# Autodesk Inventor assembly: Pump_V3
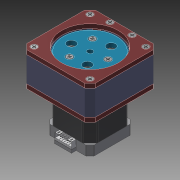
[picture p0: Inventor's stored thumbnail of the model, 180x180]
Saved by Autodesk Inventor 2022 (Build 260153000, 153)
## iProperties
Created: 2025-01-26
Part Number: Pump_V3
Document SubType Name: Assembly
Designer: Ivan
Author: Ivan
## Documents named in this file (11)
- E:\4. Прочее\1517\Предпрофессиональная олимпиада\Насос\Itteration_4\Pump_V4.iam
- E:\4. Прочее\1517\Предпрофессиональная олимпиада\Насос\Itteration_4\Nema_17.ipt
- E:\4. Прочее\1517\Предпрофессиональная олимпиада\Насос\Itteration_4\Pump_V3_Основание.ipt
- E:\4. Прочее\1517\Предпрофессиональная олимпиада\Насос\Itteration_4\ISO 7046-1 - M3 x 8_ - 4.8 - H - ISO.ipt
- E:\4. Прочее\1517\Предпрофессиональная олимпиада\Насос\Itteration_4\Pump_V3_Полумуфта.ipt
- E:\4. Прочее\1517\Предпрофессиональная олимпиада\Насос\Itteration_4\Abec 7 608 zz.ipt
- E:\4. Прочее\1517\Предпрофессиональная олимпиада\Насос\Itteration_4\Pump_V3_Втулка.ipt
- E:\4. Прочее\1517\Предпрофессиональная олимпиада\Насос\Itteration_4\Втулка Впаиваемая М3х4.2х5.ipt
- E:\4. Прочее\1517\Предпрофессиональная олимпиада\Насос\Itteration_4\ISO 7046-1 - M3 x 20_ - 4.8 - H - ISO.ipt
- E:\4. Прочее\1517\Предпрофессиональная олимпиада\Насос\Itteration_4\Pump_V4_Корпус.iam
- E:\4. Прочее\1517\Предпрофессиональная олимпиада\Насос\Itteration_4\Pump_V4_Крышка.ipt
## Components (34 placed, 10 different names)
1. Nema_17:1 — Совмещение:1, Совмещение:2, Совмещение:3, Совмещение:5
2. Pump_V3_Основание:1 — Совмещение:1, Совмещение:2, Совмещение:3, Совмещение:4, Заподлицо:1, Совмещение:6, Совмещение:15, Совмещение:16, Совмещение:17, Совмещение:21, Заподлицо:4, Совмещение:22, Совмещение:23, Совмещение:24, Заподлицо:5, Заподлицо:6, Заподлицо:7
3. Pump_V3_Полумуфта:1 — Совмещение:5, Совмещение:6, Совмещение:7, Совмещение:8, Совмещение:9, Совмещение:10, Совмещение:13, Заподлицо:2, Совмещение:14, Заподлицо:3
4. Pump_V4_Корпус:2 [sub-assembly] — Совмещение:15, Совмещение:16, Совмещение:17, Совмещение:18, Совмещение:19, Совмещение:20
5. Pump_V4_Крышка:1 — Совмещение:18, Совмещение:19, Совмещение:20, Совмещение:25, Совмещение:26, Совмещение:27, Заподлицо:8, Заподлицо:9, Заподлицо:10, Совмещение:28, Совмещение:29, Совмещение:30, Заподлицо:11, Заподлицо:12, Заподлицо:13
6. ISO 7046-1 H M3 x 8 - 4.8 - H:6 — Совмещение:26, Заподлицо:9
7. ISO 7046-1 H M3 x 8 - 4.8 - H:7 — Совмещение:25, Заподлицо:8
8. ISO 7046-1 H M3 x 8 - 4.8 - H:8 — Совмещение:21, Заподлицо:4
9. ISO 7046-1 H M3 x 8 - 4.8 - H:9 — Совмещение:27, Заподлицо:10
10. ISO 7046-1 H M3 x 8 - 4.8 - H:10 — Совмещение:24, Заподлицо:5
11. ISO 7046-1 H M3 x 8 - 4.8 - H:11 — Совмещение:22, Заподлицо:6
12. ISO 7046-1 H M3 x 8 - 4.8 - H:12 — Совмещение:23, Заподлицо:7
13. ISO 7046-1 H M3 x 8 - 4.8 - H:13 — Совмещение:28, Заподлицо:12
14. ISO 7046-1 H M3 x 8 - 4.8 - H:14 — Совмещение:29, Заподлицо:13
15. ISO 7046-1 H M3 x 8 - 4.8 - H:15 — Совмещение:30, Заподлицо:11
16. ISO 7046-1 H M3 x 8 - 4.8 - H:2 — Совмещение:4, Заподлицо:1
17. ISO 7046-1 H M3 x 8 - 4.8 - H:3
18. ISO 7046-1 H M3 x 8 - 4.8 - H:4
19. ISO 7046-1 H M3 x 8 - 4.8 - H:5
20. Abec 7 608 zz:1 — Совмещение:7, Совмещение:10, Совмещение:11
21. Abec 7 608 zz:2 — Совмещение:8, Совмещение:9, Совмещение:12
22. Pump_V3_Втулка:1 — Совмещение:11, Совмещение:12
23. Abec 7 608 zz:3
24. Abec 7 608 zz:4
25. Pump_V3_Втулка:2
26. Abec 7 608 zz:5
27. Abec 7 608 zz:6
28. Pump_V3_Втулка:3
29. Втулка Впаиваемая М3х4.2х5:1 — Совмещение:13, Заподлицо:2
30. ISO 7046-1 H M3 x 20 - 4.8 - H:2 — Совмещение:14, Заподлицо:3
31. Втулка Впаиваемая М3х4.2х5:2
32. ISO 7046-1 H M3 x 20 - 4.8 - H:3
33. Втулка Впаиваемая М3х4.2х5:3
34. ISO 7046-1 H M3 x 20 - 4.8 - H:4
## Component patterns: (4 elements, first: ISO 7046-1 H M3 x 8 - 4.8 - H:2), (3 elements, first: Abec 7 608 zz:1 + Abec 7 608 zz:2 + Pump_V3_Втулка:1), (3 elements, first: Втулка Впаиваемая М3х4.2х5:1 + ISO 7046-1 H M3 x 20 - 4.8 - H:2)
## Relationships (43: Mate 30, Flush 13)
- Совмещение:1 [Mate]: Nema_17:1 ↔ Pump_V3_Основание:1
- Совмещение:2 [Mate]: Nema_17:1 ↔ Pump_V3_Основание:1
- Совмещение:3 [Mate]: Nema_17:1 ↔ Pump_V3_Основание:1
- Совмещение:4 [Mate]: Pump_V3_Основание:1 ↔ ISO 7046-1 H M3 x 8 - 4.8 - H:2
- Заподлицо:1 [Flush]: Pump_V3_Основание:1 ↔ ISO 7046-1 H M3 x 8 - 4.8 - H:2
- Совмещение:5 [Mate]: Nema_17:1 ↔ Pump_V3_Полумуфта:1
- Совмещение:6 [Mate]: Pump_V3_Основание:1 ↔ Pump_V3_Полумуфта:1
- Совмещение:7 [Mate]: Pump_V3_Полумуфта:1 ↔ Abec 7 608 zz:1
- Совмещение:8 [Mate]: Pump_V3_Полумуфта:1 ↔ Abec 7 608 zz:2
- Совмещение:9 [Mate]: Pump_V3_Полумуфта:1 ↔ Abec 7 608 zz:2
- Совмещение:10 [Mate]: Pump_V3_Полумуфта:1 ↔ Abec 7 608 zz:1
- Совмещение:11 [Mate]: Abec 7 608 zz:1 ↔ Pump_V3_Втулка:1
- Совмещение:12 [Mate]: Abec 7 608 zz:2 ↔ Pump_V3_Втулка:1
- Совмещение:13 [Mate]: Pump_V3_Полумуфта:1 ↔ Втулка Впаиваемая М3х4.2х5:1
- Заподлицо:2 [Flush]: Pump_V3_Полумуфта:1 ↔ Втулка Впаиваемая М3х4.2х5:1
- Совмещение:14 [Mate]: Pump_V3_Полумуфта:1 ↔ ISO 7046-1 H M3 x 20 - 4.8 - H:2
- Заподлицо:3 [Flush]: Pump_V3_Полумуфта:1 ↔ ISO 7046-1 H M3 x 20 - 4.8 - H:2
- Совмещение:15 [Mate]: Pump_V3_Основание:1 ↔ Pump_V4_Корпус:2
- Совмещение:16 [Mate]: Pump_V3_Основание:1 ↔ Pump_V4_Корпус:2
- Совмещение:17 [Mate]: Pump_V3_Основание:1 ↔ Pump_V4_Корпус:2
- Совмещение:18 [Mate]: Pump_V4_Корпус:2 ↔ Pump_V4_Крышка:1
- Совмещение:19 [Mate]: Pump_V4_Корпус:2 ↔ Pump_V4_Крышка:1
- Совмещение:20 [Mate]: Pump_V4_Корпус:2 ↔ Pump_V4_Крышка:1
- Совмещение:21 [Mate]: Pump_V3_Основание:1 ↔ ISO 7046-1 H M3 x 8 - 4.8 - H:8
- Заподлицо:4 [Flush]: Pump_V3_Основание:1 ↔ ISO 7046-1 H M3 x 8 - 4.8 - H:8
- Совмещение:22 [Mate]: Pump_V3_Основание:1 ↔ ISO 7046-1 H M3 x 8 - 4.8 - H:11
- Совмещение:23 [Mate]: Pump_V3_Основание:1 ↔ ISO 7046-1 H M3 x 8 - 4.8 - H:12
- Совмещение:24 [Mate]: Pump_V3_Основание:1 ↔ ISO 7046-1 H M3 x 8 - 4.8 - H:10
- Заподлицо:5 [Flush]: Pump_V3_Основание:1 ↔ ISO 7046-1 H M3 x 8 - 4.8 - H:10
- Заподлицо:6 [Flush]: Pump_V3_Основание:1 ↔ ISO 7046-1 H M3 x 8 - 4.8 - H:11
- Заподлицо:7 [Flush]: Pump_V3_Основание:1 ↔ ISO 7046-1 H M3 x 8 - 4.8 - H:12
- Совмещение:25 [Mate]: Pump_V4_Крышка:1 ↔ ISO 7046-1 H M3 x 8 - 4.8 - H:7
- Совмещение:26 [Mate]: Pump_V4_Крышка:1 ↔ ISO 7046-1 H M3 x 8 - 4.8 - H:6
- Совмещение:27 [Mate]: Pump_V4_Крышка:1 ↔ ISO 7046-1 H M3 x 8 - 4.8 - H:9
- Заподлицо:8 [Flush]: Pump_V4_Крышка:1 ↔ ISO 7046-1 H M3 x 8 - 4.8 - H:7
- Заподлицо:9 [Flush]: Pump_V4_Крышка:1 ↔ ISO 7046-1 H M3 x 8 - 4.8 - H:6
- Заподлицо:10 [Flush]: Pump_V4_Крышка:1 ↔ ISO 7046-1 H M3 x 8 - 4.8 - H:9
- Совмещение:28 [Mate]: Pump_V4_Крышка:1 ↔ ISO 7046-1 H M3 x 8 - 4.8 - H:13
- Совмещение:29 [Mate]: Pump_V4_Крышка:1 ↔ ISO 7046-1 H M3 x 8 - 4.8 - H:14
- Совмещение:30 [Mate]: Pump_V4_Крышка:1 ↔ ISO 7046-1 H M3 x 8 - 4.8 - H:15
- Заподлицо:11 [Flush]: Pump_V4_Крышка:1 ↔ ISO 7046-1 H M3 x 8 - 4.8 - H:15
- Заподлицо:12 [Flush]: Pump_V4_Крышка:1 ↔ ISO 7046-1 H M3 x 8 - 4.8 - H:13
- Заподлицо:13 [Flush]: Pump_V4_Крышка:1 ↔ ISO 7046-1 H M3 x 8 - 4.8 - H:14
